# Autodesk Inventor assembly: Linear_Unit
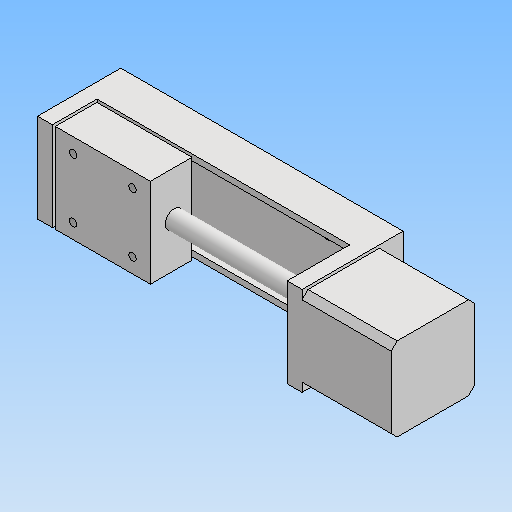
[picture p0: Inventor's stored thumbnail of the model, 512x512]
Saved by Autodesk Inventor 2020 (Build 240168000, 168)
## iProperties
Created: 2021-07-13
Part Number: Linear_Unit
Document SubType Name: Assembly
Designer: ken113
Author: ken113
## Documents named in this file (3)
- C:\Users\lvglv\Documents\GitHub\CoreXY_Laser\Model\Parts\Linear_Guide\Linear_Unit\Linear_Unit.iam
- C:\Users\lvglv\Documents\GitHub\CoreXY_Laser\Model\Parts\Linear_Guide\Linear_Unit\Linear_Unit_A.ipt
- C:\Users\lvglv\Documents\GitHub\CoreXY_Laser\Model\Parts\Linear_Guide\Linear_Unit\Linear_Unit_B.ipt
## Components (2 placed, 2 different names)
1. Linear_Unit_A:1 — メイト:1, フラッシュ:1
2. Linear_Unit_B:1 — メイト:1, フラッシュ:1
## Relationships (2: Mate 1, Flush 1)
- メイト:1 [Mate]: Linear_Unit_A:1 ↔ Linear_Unit_B:1
- フラッシュ:1 [Flush]: Linear_Unit_A:1 ↔ Linear_Unit_B:1
